# Autodesk Inventor assembly: ForearmActuatorConnector
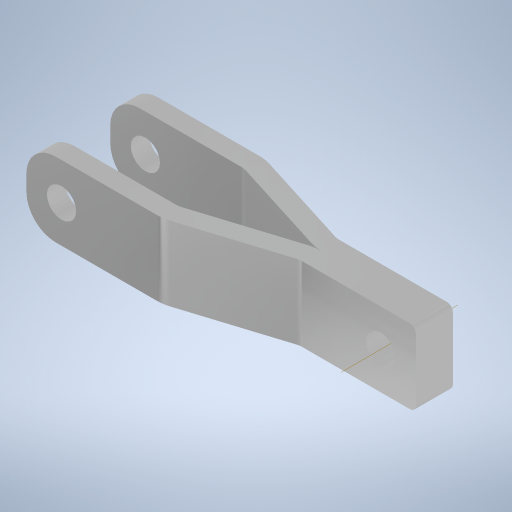
[picture p0: Inventor's stored thumbnail of the model, 512x512]
Saved by Autodesk Inventor 2023 (Build 270158000, 158)
## iProperties
Created: 2023-03-27
Part Number: ForearmActuatorConnector
Document SubType Name: Assembly
Designer: LattePanda
Author: LattePanda
## Documents named in this file (3)
- C:\Users\LattePanda\Desktop\str1ker\cad\ForearmActuatorConnector.iam
- C:\Users\LattePanda\Desktop\str1ker\cad\ForearmActuatorConnector.ipt
- C:\Users\LattePanda\Desktop\str1ker\cad\ForearmActuatorConnectorBoundingBox.ipt
## Components (3 placed, 2 different names)
1. ForearmActuatorConnector:1 — Mate:1, Mate:5, Flush:5
2. ForearmActuatorConnector:2 — Mate:3, Angle:1, Mate:4, Flush:3, Mate:5
3. ForearmActuatorConnectorBoundingBox:1 — Flush:1, Flush:3, Flush:4, Flush:5
## Relationships (9: Mate 4, Flush 4, Angle 1)
- Mate:1: ForearmActuatorConnector:1
- Mate:3: ForearmActuatorConnector:2
- Angle:1 (180 deg): ForearmActuatorConnector:2
- Mate:4: ForearmActuatorConnector:2
- Flush:1: ForearmActuatorConnectorBoundingBox:1
- Flush:3: ForearmActuatorConnector:2 ↔ ForearmActuatorConnectorBoundingBox:1
- Flush:4: ForearmActuatorConnectorBoundingBox:1
- Mate:5: ForearmActuatorConnector:1 ↔ ForearmActuatorConnector:2
- Flush:5: ForearmActuatorConnector:1 ↔ ForearmActuatorConnectorBoundingBox:1
